# Autodesk Inventor assembly: CuttingHead
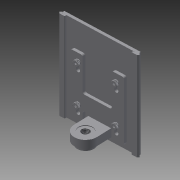
[picture p0: Inventor's stored thumbnail of the model, 180x180]
Saved by Autodesk Inventor 2013 (Build 170138000, 138)
## iProperties
Created: 2012-12-07
Part Number: CuttingHead
Document SubType Name: Assembly
Designer: istvan.burbank
Author: istvan.burbank
## Documents named in this file (8)
- D:\GitHub\Crown-Fire\CAD\Frame\CuttingHead\CuttingHead.iam
- D:\GitHub\Crown-Fire\CAD\Frame\CuttingHead\AcmeRoundNut.ipt
- D:\GitHub\Crown-Fire\CAD\Frame\CuttingHead\AcmeMountingFlange.ipt
- D:\GitHub\Crown-Fire\CAD\Frame\CuttingHead\backPlate.ipt
- D:\GitHub\Crown-Fire\CAD\Frame\CuttingHead\vee-track.ipt
- D:\GitHub\Crown-Fire\CAD\Templates\vee-track.ipt
- D:\GitHub\Crown-Fire\CAD\Frame\CuttingHead\torchMount_back.ipt
- D:\GitHub\Crown-Fire\CAD\Hardware\z-axisSliderShoulderBolts.ipt
## Components (10 placed, 6 different names)
1. AcmeRoundNut:1 — Mate:1, Mate:2
2. AcmeMountingFlange:1 — Mate:1, Mate:2, Mate:3, Flush:3
3. backPlate:1 — Mate:3, Mate:4, Mate:5, Mate:6, Mate:7, Flush:1, Flush:2, Flush:3, Mate:8, Mate:9, Mate:10, Mate:11, Mate:12
4. vee-track:1 — Mate:4, Mate:7, Flush:1
5. vee-track:2 — Mate:5, Mate:6, Flush:2
6. torchMount_back:1 — Tangent:1, Tangent:2, Mate:12, Mate:13, Mate:14, Mate:15, Mate:16
7. z-axisSliderShoulderBolts:1 — Mate:8, Tangent:1, Mate:13
8. z-axisSliderShoulderBolts:2 — Mate:9, Mate:14
9. z-axisSliderShoulderBolts:3 — Mate:10, Tangent:2, Mate:15
10. z-axisSliderShoulderBolts:4 — Mate:11, Mate:16
## Relationships (21: Mate 16, Flush 3, Tangent 2)
- Mate:1: AcmeRoundNut:1 ↔ AcmeMountingFlange:1
- Mate:2: AcmeRoundNut:1 ↔ AcmeMountingFlange:1
- Mate:3: AcmeMountingFlange:1 ↔ backPlate:1
- Mate:4: backPlate:1 ↔ vee-track:1
- Mate:5: backPlate:1 ↔ vee-track:2
- Mate:6: backPlate:1 ↔ vee-track:2
- Mate:7: backPlate:1 ↔ vee-track:1
- Flush:1: backPlate:1 ↔ vee-track:1
- Flush:2: backPlate:1 ↔ vee-track:2
- Flush:3 (-6.35 mm): AcmeMountingFlange:1 ↔ backPlate:1
- Mate:8: backPlate:1 ↔ z-axisSliderShoulderBolts:1
- Mate:9: backPlate:1 ↔ z-axisSliderShoulderBolts:2
- Mate:10: backPlate:1 ↔ z-axisSliderShoulderBolts:3
- Mate:11: backPlate:1 ↔ z-axisSliderShoulderBolts:4
- Tangent:1: torchMount_back:1 ↔ z-axisSliderShoulderBolts:1
- Tangent:2: torchMount_back:1 ↔ z-axisSliderShoulderBolts:3
- Mate:12: backPlate:1 ↔ torchMount_back:1
- Mate:13: torchMount_back:1 ↔ z-axisSliderShoulderBolts:1
- Mate:14: torchMount_back:1 ↔ z-axisSliderShoulderBolts:2
- Mate:15: torchMount_back:1 ↔ z-axisSliderShoulderBolts:3
- Mate:16: torchMount_back:1 ↔ z-axisSliderShoulderBolts:4
